# Autodesk Inventor assembly: Subensamble_cortadora
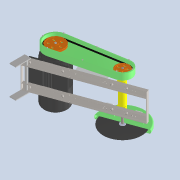
[picture p0: Inventor's stored thumbnail of the model, 180x180]
Saved by Autodesk Inventor 2021 (Build 250183000, 183)
## iProperties
Created: 2009-02-21
Part Number: Subensamble_cortadora
Document SubType Name: Assembly
Designer: Admin
Sending System: SolidWorks 2010
Last Author: Dominic
Last Saved: 2012-06-29
Author: Admin
## Documents named in this file (4)
- C:\Users\Admin\OneDrive - Universidad Nacional de Colombia\Doceabo semestre\AUTO\proyecto Auto\Proyecto_APM\CADs estaciones a automatizar\Estación corte\Subensamble_cortadora.iam
- C:\Users\Admin\OneDrive - Universidad Nacional de Colombia\Doceabo semestre\AUTO\proyecto Auto\Proyecto_APM\CADs estaciones a automatizar\Estación corte\belt cover lid.ipt
- C:\Users\Admin\OneDrive - Universidad Nacional de Colombia\Doceabo semestre\AUTO\proyecto Auto\Proyecto_APM\CADs estaciones a automatizar\Estación corte\Grupo_cortadora.iam
- C:\Users\Admin\OneDrive - Universidad Nacional de Colombia\Doceabo semestre\AUTO\proyecto Auto\Proyecto_APM\CADs estaciones a automatizar\Estación corte\Subensamble_Base cortadora.iam
## Components (3 placed, 3 different names)
1. belt cover lid:3
2. Grupo_cortadora:1 [sub-assembly] — De rotación:1
3. Subensamble_Base cortadora:1 [sub-assembly] — De rotación:1
## Relationships (1: RevoluteJoint 1)
- De rotación:1 [RevoluteJoint] (0.05 mm): Grupo_cortadora:1 ↔ Subensamble_Base cortadora:1
